# Autodesk Inventor assembly: Assembly
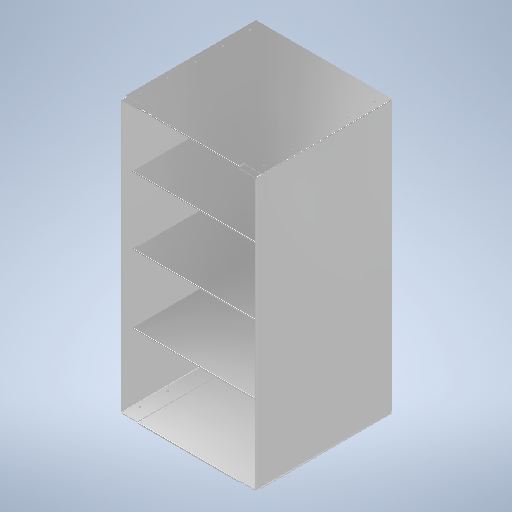
[picture p0: Inventor's stored thumbnail of the model, 512x512]
Saved by Autodesk Inventor 2025.2 (Build 292293000, 293)
## iProperties
Created: 2025-03-19
Part Number: Assembly
Document SubType Name: Assembly
Designer: bless
Author: bless
## Documents named in this file (8)
- C:\Users\bless\OneDrive - Conestoga College\Documents\Inventor\8071W25\Assignment\Assembly.iam
- C:\Users\bless\OneDrive - Conestoga College\Documents\Inventor\8071W25\Assignment\left side.ipt
- C:\Users\bless\OneDrive - Conestoga College\Documents\Inventor\8071W25\Assignment\left side_MIR.ipt
- C:\Users\bless\OneDrive - Conestoga College\Documents\Inventor\8071W25\Assignment\top.ipt
- C:\Users\bless\OneDrive - Conestoga College\Documents\Inventor\8071W25\Assignment\top_MIR.ipt
- C:\Users\bless\OneDrive - Conestoga College\Documents\Inventor\8071W25\Assignment\shelves.ipt
- C:\Users\bless\OneDrive - Conestoga College\Documents\Inventor\8071W25\Assignment\shelves_MIR.ipt
- C:\Users\bless\OneDrive - Conestoga College\Documents\Inventor\8071W25\Assignment\shelves_MIR1.ipt
## Components (7 placed, 7 different names)
1. left side:1 — Flush:1, Flush:2
2. left side_MIR:1 — Mate:1
3. top:1 — Flush:2, Flush:3, Flush:4
4. top_MIR:1 — Mate:2, Flush:5
5. shelves:1 — Flush:4, Flush:5, Flush:6, Flush:7
6. shelves_MIR:1 — Mate:3
7. shelves_MIR1:1 — Flush:8, Mate:4
## Relationships (12: Flush 8, Mate 4)
- Flush:1 (-304.8 mm): left side:1
- Mate:1 (-304.8 mm): left side_MIR:1
- Flush:2: left side:1 ↔ top:1
- Flush:3 (-612.775 mm): top:1
- Mate:2 (-612.775 mm): top_MIR:1
- Flush:4: top:1 ↔ shelves:1
- Flush:5 (-611.2002 mm): top_MIR:1 ↔ shelves:1
- Flush:6 (152.3873 mm): shelves:1
- Mate:3 (149.2123 mm): shelves_MIR:1
- Flush:7 (-153.9875 mm): shelves:1
- Flush:8 (152.3873 mm): shelves_MIR1:1
- Mate:4 (-153.9875 mm): shelves_MIR1:1
